# Autodesk Inventor assembly: design 1
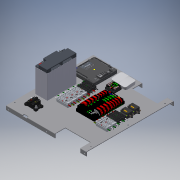
[picture p0: Inventor's stored thumbnail of the model, 180x180]
Saved by Autodesk Inventor 2016 (Build 200138000, 138)
## iProperties
Created: 2017-01-22
Part Number: design 1
Document SubType Name: Assembly
Designer: Taylor Goyette
Author: Taylor Goyette
## Documents named in this file (11)
- C:\Users\Kyle\Documents\FRC1073\Robot2017\DriveTrain\Belly pan with electronics\design 1.iam
- C:\Users\Kyle\Documents\FRC1073\Robot2017\DriveTrain\BellyPan2.ipt
- C:\Users\Kyle\Documents\FRC1073\Robot2017\DriveTrain\Belly pan with electronics\FRC KOP 2016\Electrical\ELEC_CircuitBreaker_CB185-120.iam
- C:\Users\Kyle\Documents\FRC1073\Robot2017\DriveTrain\Belly pan with electronics\FRC KOP 2016\Electrical\fc16-024_VoltRegModule.ipt
- C:\Users\Kyle\Documents\FRC1073\Robot2017\DriveTrain\Belly pan with electronics\FRC KOP 2016\Electrical\fc16-036_Battery.iam
- C:\Users\Kyle\Documents\FRC1073\Robot2017\DriveTrain\Belly pan with electronics\FRC KOP 2016\Control System\CS_Controller_ROBORIO.ipt
- C:\Users\Kyle\Documents\FRC1073\Robot2017\DriveTrain\Belly pan with electronics\FRC KOP 2016\Control System\CS_DistrPanel_14-806880.ipt
- C:\Users\Kyle\Documents\FRC1073\Robot2017\DriveTrain\Belly pan with electronics\FRC KOP 2016\Control System\CS_Controller_217-8080.ipt
- C:\Users\Kyle\Documents\FRC1073\Robot2017\DriveTrain\Belly pan with electronics\FRC KOP 2016\OM5P-AN.ipt
- C:\Users\Kyle\Documents\FRC1073\Robot2017\DriveTrain\Belly pan with electronics\FRC KOP 2016\spike relay.ipt
- C:\Users\Kyle\Documents\FRC1073\Robot2017\DriveTrain\Belly pan with electronics\FRC KOP 2016\Control System\CS_Controller_217-9090.ipt
## Components (19 placed, 10 different names)
1. BellyPan2:1 — Mate:2, Mate:3, Flush:1, Mate:14, Mate:16, Flush:18, Mate:19, Mate:20, Mate:22
2. ELEC_CircuitBreaker_CB185-120:1 [sub-assembly] — Mate:19, Mate:20
3. fc16-024_VoltRegModule:1 — Mate:14
4. fc16-036_Battery:1 [sub-assembly] — Mate:3, Flush:1
5. CS_Controller_ROBORIO:1 — Mate:16, Flush:18, Flush:19
6. CS_DistrPanel_14-806880:1 — Mate:2
7. OM5P-AN:1 — Flush:19
8. spike relay:1
9. spike relay:2
10. CS_Controller_217-8080:7 — Flush:21, Flush:22, Flush:24, Flush:25
11. CS_Controller_217-8080:8 — Flush:21, Flush:22
12. CS_Controller_217-9090:2 — Flush:23, Flush:24, Flush:26
13. CS_Controller_217-9090:3 — Flush:23, Flush:25, Flush:26
14. CS_Controller_217-8080:9 — Flush:31, Flush:32, Flush:34
15. CS_Controller_217-8080:10 — Mate:22, Flush:31
16. CS_Controller_217-9090:4 — Flush:27, Flush:35, Mate:24
17. CS_Controller_217-9090:5 — Flush:27, Mate:24
18. CS_Controller_217-8080:11 — Flush:32, Flush:34
19. CS_Controller_217-8080:12 — Flush:35
## Relationships (22: Flush 14, Mate 8)
- Mate:2: BellyPan2:1 ↔ CS_DistrPanel_14-806880:1
- Mate:3: BellyPan2:1 ↔ fc16-036_Battery:1
- Flush:1 (28.575 mm): BellyPan2:1 ↔ fc16-036_Battery:1
- Mate:14: BellyPan2:1 ↔ fc16-024_VoltRegModule:1
- Mate:16: BellyPan2:1 ↔ CS_Controller_ROBORIO:1
- Flush:18 (25.4 mm): BellyPan2:1 ↔ CS_Controller_ROBORIO:1
- Flush:19: CS_Controller_ROBORIO:1 ↔ OM5P-AN:1
- Flush:21: CS_Controller_217-8080:7 ↔ CS_Controller_217-8080:8
- Flush:22: CS_Controller_217-8080:7 ↔ CS_Controller_217-8080:8
- Mate:19: BellyPan2:1 ↔ ELEC_CircuitBreaker_CB185-120:1
- Mate:20: BellyPan2:1 ↔ ELEC_CircuitBreaker_CB185-120:1
- Flush:23: CS_Controller_217-9090:2 ↔ CS_Controller_217-9090:3
- Flush:24: CS_Controller_217-8080:7 ↔ CS_Controller_217-9090:2
- Flush:25: CS_Controller_217-8080:7 ↔ CS_Controller_217-9090:3
- Flush:26: CS_Controller_217-9090:2 ↔ CS_Controller_217-9090:3
- Flush:27: CS_Controller_217-9090:4 ↔ CS_Controller_217-9090:5
- Mate:22: BellyPan2:1 ↔ CS_Controller_217-8080:10
- Flush:31: CS_Controller_217-8080:9 ↔ CS_Controller_217-8080:10
- Flush:32: CS_Controller_217-8080:9 ↔ CS_Controller_217-8080:11
- Flush:34: CS_Controller_217-8080:9 ↔ CS_Controller_217-8080:11
- Flush:35: CS_Controller_217-9090:4 ↔ CS_Controller_217-8080:12
- Mate:24 (1.1684 mm): CS_Controller_217-9090:4 ↔ CS_Controller_217-9090:5
